# Autodesk Inventor assembly: KabineChassis
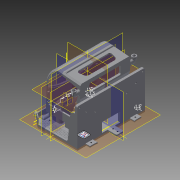
[picture p0: Inventor's stored thumbnail of the model, 180x180]
Saved by Autodesk Inventor 2015 (Build 190159000, 159)
## iProperties
Created: 2018-10-29
Part Number: KabineChassis
Document SubType Name: Assembly
Designer: Boris
Author: Boris
## Documents named in this file (8)
- D:\Wisag Hiserv\HiSERV Smart Drive\WorkOrder\3D - Teile\KabineChassis.iam
- D:\Wisag Hiserv\HiSERV Smart Drive\WorkOrder\3D - Teile\KabineChassis.ipt
- D:\Wisag Hiserv\HiSERV Smart Drive\WorkOrder\3D - Teile\Lenkrad.ipt
- D:\Wisag Hiserv\HiSERV Smart Drive\WorkOrder\3D - Teile\KabineTeil1.ipt
- D:\Wisag Hiserv\HiSERV Smart Drive\WorkOrder\3D - Teile\ScheinwerferFront.ipt
- D:\Wisag Hiserv\HiSERV Smart Drive\WorkOrder\3D - Teile\SchleppstangeBefestigung.ipt
- D:\Wisag Hiserv\HiSERV Smart Drive\WorkOrder\3D - Teile\SchleppstangeBefestigungOben.ipt
- D:\Wisag Hiserv\HiSERV Smart Drive\WorkOrder\3D - Teile\SchleppstangeBefestigungUnten.ipt
## Components (8 placed, 7 different names)
1. KabineChassis:1 — Einfügen:2, Einfügen:3, Einfügen:4, Einfügen:5, Einfügen:6, Einfügen:7
2. Lenkrad:1 — Einfügen:2
3. KabineTeil1:1 — Einfügen:3
4. ScheinwerferFront:1 — Einfügen:4
5. ScheinwerferFront:2 — Einfügen:5
6. SchleppstangeBefestigung:1 — Einfügen:7, Einfügen:8
7. SchleppstangeBefestigungOben:1 — Einfügen:8
8. SchleppstangeBefestigungUnten:1 — Einfügen:6
## Relationships (7: Insert 7)
- Einfügen:2 [Insert] (-2.5 mm): KabineChassis:1 ↔ Lenkrad:1
- Einfügen:3 [Insert] (10 mm): KabineChassis:1 ↔ KabineTeil1:1
- Einfügen:4 [Insert] (-5 mm): KabineChassis:1 ↔ ScheinwerferFront:1
- Einfügen:5 [Insert] (-10 mm): KabineChassis:1 ↔ ScheinwerferFront:2
- Einfügen:6 [Insert] (5 mm): KabineChassis:1 ↔ SchleppstangeBefestigungUnten:1
- Einfügen:7 [Insert]: KabineChassis:1 ↔ SchleppstangeBefestigung:1
- Einfügen:8 [Insert] (3 mm): SchleppstangeBefestigung:1 ↔ SchleppstangeBefestigungOben:1
